# Autodesk Inventor assembly: 电路装配
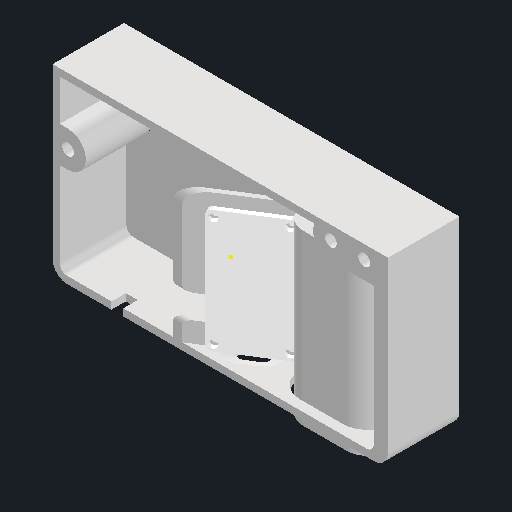
[picture p0: Inventor's stored thumbnail of the model, 512x512]
Saved by Autodesk Inventor 2025 (Build 290162000, 162)
## iProperties
Created: 2026-03-02
Part Number: 电路装配
Document SubType Name: Assembly
Designer: XH
Author: XH
## Documents named in this file (4)
- C:\1A_Engineering_files\braille-printer-v2\3D文件\电路装配.iam
- C:\1A_Engineering_files\braille-printer-v2\3D文件\ESP32.ipt
- C:\1A_Engineering_files\braille-printer-v2\3D文件\后盖电路.ipt
- C:\1A_Engineering_files\braille-printer-v2\3D文件\电池.ipt
## Components (3 placed, 3 different names)
1. ESP32:1 — 配合:4, 配合:5
2. 后盖电路:1 — 配合:2, 配合:4, 配合:5
3. 电池:1 — 配合:2
## Relationships (3: Mate 3)
- 配合:2 [Mate]: 后盖电路:1 ↔ 电池:1
- 配合:4 [Mate]: ESP32:1 ↔ 后盖电路:1
- 配合:5 [Mate]: ESP32:1 ↔ 后盖电路:1
